# Autodesk Inventor assembly: ControllerMount
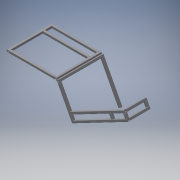
[picture p0: Inventor's stored thumbnail of the model, 180x180]
Saved by Autodesk Inventor 2016 (Build 200138000, 138)
## iProperties
Created: 2016-06-23
Part Number: ControllerMount
Document SubType Name: Assembly
Designer: cutrones
Author: cutrones
## Documents named in this file (9)
- C:\Users\cutrones\Desktop\motionbase\CAD\MotionBaseCAD\ControllerMount\ControllerMount.iam
- C:\Users\cutrones\Desktop\motionbase\CAD\MotionBaseCAD\ControllerMount\InitialVert.ipt
- C:\Users\cutrones\Desktop\motionbase\CAD\MotionBaseCAD\ControllerMount\2ndVert.ipt
- C:\Users\cutrones\Desktop\motionbase\CAD\MotionBaseCAD\ControllerMount\InitialHoriz.ipt
- C:\Users\cutrones\Desktop\motionbase\CAD\MotionBaseCAD\ControllerMount\FrontHoriz.ipt
- C:\Users\cutrones\Desktop\motionbase\CAD\MotionBaseCAD\ControllerMount\LegExtrusion.ipt
- C:\Users\cutrones\Desktop\motionbase\CAD\MotionBaseCAD\ControllerMount\LegBracing.ipt
- C:\Users\cutrones\Desktop\motionbase\CAD\MotionBaseCAD\ControllerMount\HeelBar.ipt
- C:\Users\cutrones\Desktop\motionbase\CAD\MotionBaseCAD\ControllerMount\FrontHorizTop.ipt
## Components (15 placed, 8 different names)
1. InitialVert:1 — Mate:1, Mate:2, Mate:3, Flush:1, Flush:2, Flush:5, Flush:7, Flush:10, Mate:8
2. 2ndVert:1 — Flush:1, Flush:2, Mate:4, Flush:3, Flush:8, Mate:6, Mate:7, Flush:9, Flush:11, Tangent:1
3. InitialHoriz:1 — Mate:4, Flush:3, Flush:5, Mate:8
4. InitialHoriz:3 — Flush:7, Flush:8, Mate:6
5. InitialHoriz:4 — Mate:7, Flush:9, Flush:10
6. 2ndVert:2 — Flush:11, Tangent:1, Mate:11, Flush:16, Flush:19, Mate:22, Flush:37, Flush:38
7. FrontHoriz:1 — Mate:11, Flush:16, Flush:19, Mate:13, Flush:20, Mate:14, Flush:21, Flush:36
8. LegExtrusion:1 — Mate:13, Flush:20, Flush:30, Flush:31, Mate:18, Mate:21, Flush:36
9. LegExtrusion:2 — Mate:14, Flush:21, Mate:15, Flush:24, Flush:25, Mate:16, Flush:26, Flush:32, Mate:19, Flush:33
10. LegBracing:2 — Mate:16, Flush:26, Flush:28, Mate:21
11. LegBracing:3 — Mate:15, Flush:24, Flush:25, Flush:28
12. HeelBar:1 — Flush:32, Mate:19, Flush:33, Flush:35, Mate:20
13. HeelBar:2 — Flush:30, Flush:31, Mate:18, Flush:34
14. LegBracing:4 — Flush:34, Flush:35, Mate:20
15. FrontHorizTop:1 — Mate:22, Flush:37, Flush:38
## Relationships (44: Flush 26, Mate 17, Tangent 1)
- Mate:1: InitialVert:1
- Mate:2: InitialVert:1
- Mate:3: InitialVert:1
- Flush:1: InitialVert:1 ↔ 2ndVert:1
- Flush:2: InitialVert:1 ↔ 2ndVert:1
- Mate:4: 2ndVert:1 ↔ InitialHoriz:1
- Flush:3: 2ndVert:1 ↔ InitialHoriz:1
- Flush:5 (-101.6 mm): InitialVert:1 ↔ InitialHoriz:1
- Flush:7: InitialVert:1 ↔ InitialHoriz:3
- Flush:8: 2ndVert:1 ↔ InitialHoriz:3
- Mate:6: 2ndVert:1 ↔ InitialHoriz:3
- Mate:7: 2ndVert:1 ↔ InitialHoriz:4
- Flush:9: 2ndVert:1 ↔ InitialHoriz:4
- Flush:10: InitialVert:1 ↔ InitialHoriz:4
- Mate:8: InitialVert:1 ↔ InitialHoriz:1
- Flush:11: 2ndVert:1 ↔ 2ndVert:2
- Tangent:1: 2ndVert:1 ↔ 2ndVert:2
- Mate:11: 2ndVert:2 ↔ FrontHoriz:1
- Flush:16: 2ndVert:2 ↔ FrontHoriz:1
- Flush:19: 2ndVert:2 ↔ FrontHoriz:1
- Mate:13: FrontHoriz:1 ↔ LegExtrusion:1
- Flush:20: FrontHoriz:1 ↔ LegExtrusion:1
- Mate:14: FrontHoriz:1 ↔ LegExtrusion:2
- Flush:21: FrontHoriz:1 ↔ LegExtrusion:2
- Mate:15: LegExtrusion:2 ↔ LegBracing:3
- Flush:24: LegExtrusion:2 ↔ LegBracing:3
- Flush:25: LegExtrusion:2 ↔ LegBracing:3
- Mate:16: LegExtrusion:2 ↔ LegBracing:2
- Flush:26: LegExtrusion:2 ↔ LegBracing:2
- Flush:28 (177.8 mm): LegBracing:2 ↔ LegBracing:3
- Flush:30: LegExtrusion:1 ↔ HeelBar:2
- Flush:31: LegExtrusion:1 ↔ HeelBar:2
- Mate:18: LegExtrusion:1 ↔ HeelBar:2
- Flush:32: LegExtrusion:2 ↔ HeelBar:1
- Mate:19: LegExtrusion:2 ↔ HeelBar:1
- Flush:33: LegExtrusion:2 ↔ HeelBar:1
- Flush:34: HeelBar:2 ↔ LegBracing:4
- Flush:35: HeelBar:1 ↔ LegBracing:4
- Mate:20: HeelBar:1 ↔ LegBracing:4
- Mate:21: LegExtrusion:1 ↔ LegBracing:2
- Flush:36: FrontHoriz:1 ↔ LegExtrusion:1
- Mate:22: 2ndVert:2 ↔ FrontHorizTop:1
- Flush:37: 2ndVert:2 ↔ FrontHorizTop:1
- Flush:38: 2ndVert:2 ↔ FrontHorizTop:1
